# Autodesk Inventor assembly: SolderSupport
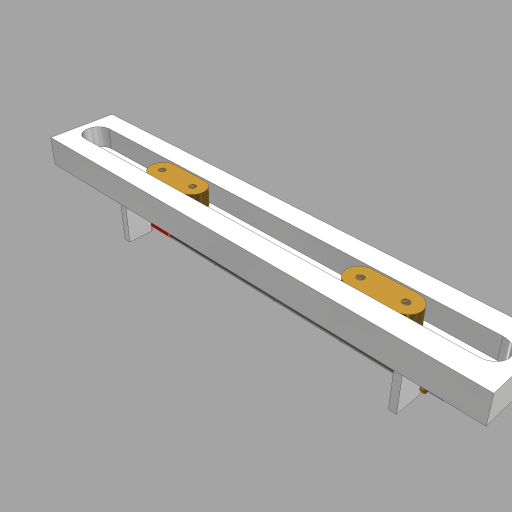
[picture p0: Inventor's stored thumbnail of the model, 512x512]
Saved by Autodesk Inventor 2024 (Build 280153020, 153B)
## iProperties
Created: 2023-09-27
Part Number: SolderSupport
Document SubType Name: Assembly
Designer: schanen
Author: schanen
## Documents named in this file (8)
- C:\Users\schanen\Documents\Inventor\he4inserts\SolderSupport.iam
- C:\Users\schanen\Documents\Inventor\he4inserts\CompositeSupport-3.iam
- C:\Users\schanen\Documents\Inventor\he4inserts\SupportSlide.ipt
- C:\Users\schanen\Documents\Inventor\he4inserts\SolderSupport.ipt
- C:\Users\schanen\Documents\Inventor\he4inserts\Screw_StainlessSteal_M3_SocketCap_6mm.ipt
- C:\Users\schanen\Documents\Inventor\he4inserts\SolderSupportDoubleNut.ipt
- C:\Users\schanen\Documents\Inventor\he4inserts\Screw_StainlessSteal_M2_SocketCap_10mm.ipt
- C:\Users\schanen\Documents\Inventor\he4inserts\Nut_M2_Brass.ipt
## Components (12 placed, 7 different names)
1. CompositeSupport-3:1 [sub-assembly] — Mate:2, Mate:4, Mate:13, Mate:26, Mate:28
2. SupportSlide:1 — Mate:2, Mate:5, Mate:6, Mate:11, Mate:12, Mate:13, Mate:24, Mate:25, Mate:29
3. SolderSupport:1 — Mate:14, Mate:19, Mate:20, Mate:21, Mate:22, Mate:23, Mate:24, Mate:25
4. SupportSlide:2 — Mate:4, Mate:7, Mate:8, Mate:9, Mate:10, Mate:22, Mate:23, Mate:27
5. Screw_StainlessSteal_M3_SocketCap_6mm:1 — Mate:5, Mate:11, Mate:16
6. Screw_StainlessSteal_M3_SocketCap_6mm:2 — Mate:6, Mate:12, Mate:17
7. Screw_StainlessSteal_M3_SocketCap_6mm:3 — Mate:7, Mate:9, Mate:18
8. Screw_StainlessSteal_M3_SocketCap_6mm:4 — Mate:8, Mate:10, Mate:15
9. SolderSupportDoubleNut:1 — Mate:15, Mate:18, Mate:19
10. SolderSupportDoubleNut:2 — Mate:16, Mate:17, Mate:20
11. Screw_StainlessSteal_M2_SocketCap_10mm:1 — Mate:26, Mate:27
12. Nut_M2_Brass:1 — Mate:28, Mate:29
## Relationships (27: Mate 27)
- Mate:2: CompositeSupport-3:1 ↔ SupportSlide:1
- Mate:4: CompositeSupport-3:1 ↔ SupportSlide:2
- Mate:5: SupportSlide:1 ↔ Screw_StainlessSteal_M3_SocketCap_6mm:1
- Mate:6: SupportSlide:1 ↔ Screw_StainlessSteal_M3_SocketCap_6mm:2
- Mate:7: SupportSlide:2 ↔ Screw_StainlessSteal_M3_SocketCap_6mm:3
- Mate:8: SupportSlide:2 ↔ Screw_StainlessSteal_M3_SocketCap_6mm:4
- Mate:9: SupportSlide:2 ↔ Screw_StainlessSteal_M3_SocketCap_6mm:3
- Mate:10: SupportSlide:2 ↔ Screw_StainlessSteal_M3_SocketCap_6mm:4
- Mate:11: SupportSlide:1 ↔ Screw_StainlessSteal_M3_SocketCap_6mm:1
- Mate:12: SupportSlide:1 ↔ Screw_StainlessSteal_M3_SocketCap_6mm:2
- Mate:13: CompositeSupport-3:1 ↔ SupportSlide:1
- Mate:14 (-15 mm): SolderSupport:1
- Mate:15: Screw_StainlessSteal_M3_SocketCap_6mm:4 ↔ SolderSupportDoubleNut:1
- Mate:16: Screw_StainlessSteal_M3_SocketCap_6mm:1 ↔ SolderSupportDoubleNut:2
- Mate:17: Screw_StainlessSteal_M3_SocketCap_6mm:2 ↔ SolderSupportDoubleNut:2
- Mate:18: Screw_StainlessSteal_M3_SocketCap_6mm:3 ↔ SolderSupportDoubleNut:1
- Mate:19: SolderSupport:1 ↔ SolderSupportDoubleNut:1
- Mate:20: SolderSupport:1 ↔ SolderSupportDoubleNut:2
- Mate:21: SolderSupport:1
- Mate:22: SolderSupport:1 ↔ SupportSlide:2
- Mate:23: SolderSupport:1 ↔ SupportSlide:2
- Mate:24: SupportSlide:1 ↔ SolderSupport:1
- Mate:25: SupportSlide:1 ↔ SolderSupport:1
- Mate:26: CompositeSupport-3:1 ↔ Screw_StainlessSteal_M2_SocketCap_10mm:1
- Mate:27: SupportSlide:2 ↔ Screw_StainlessSteal_M2_SocketCap_10mm:1
- Mate:28: CompositeSupport-3:1 ↔ Nut_M2_Brass:1
- Mate:29: SupportSlide:1 ↔ Nut_M2_Brass:1
